# Autodesk Inventor assembly: Rack
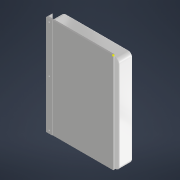
[picture p0: Inventor's stored thumbnail of the model, 180x180]
Saved by Autodesk Inventor 2021 (Build 250183000, 183)
## iProperties
Created: 2023-03-30
Part Number: Rack
Document SubType Name: Assembly
Designer: casey
Author: casey
## Documents named in this file (5)
- C:\Users\casey\Desktop\dev\Rack\Rack.iam
- C:\Users\casey\Desktop\dev\Rack\parts\box.ipt
- C:\Users\casey\Desktop\dev\Rack\parts\slide_panel.ipt
- C:\Users\casey\Desktop\dev\Rack\parts\slide_panel_fixation_angle.ipt
- C:\Users\casey\Desktop\dev\Rack\parts\slide_panel_back_stopper.ipt
## Components (4 placed, 4 different names)
1. box:1
2. slide_panel:1 — フラッシュ:1, 挿入:1
3. slide_panel_fixation_angle:1 — フラッシュ:1
4. slide_panel_back_stopper:1 — 挿入:1
## Relationships (2: Flush 1, Insert 1)
- フラッシュ:1 [Flush]: slide_panel:1 ↔ slide_panel_fixation_angle:1
- 挿入:1 [Insert]: slide_panel:1 ↔ slide_panel_back_stopper:1
